# Autodesk Inventor assembly: supportForWinch
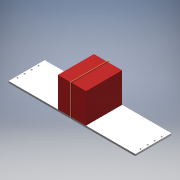
[picture p0: Inventor's stored thumbnail of the model, 180x180]
Saved by Autodesk Inventor 2018.2 (Build 222227000, 227)
## iProperties
Created: 2018-01-10
Part Number: supportForWinch
Document SubType Name: Assembly
Designer: steele
Author: steele
## Documents named in this file (3)
- D:\snobotics\CAD-Development\robSteele\2018-FRC\supportForWinch.iam
- D:\snobotics\CAD-Development\robSteele\2018-FRC\AluminumPlateForWinch.ipt
- D:\snobotics\CAD-Development\robSteele\2018-FRC\WinchVolume.ipt
## Components (2 placed, 2 different names)
1. AluminumPlateForWinch:1 — Mate:6, Flush:3
2. WinchVolume:1 — Mate:6, Flush:3
## Relationships (2: Mate 1, Flush 1)
- Mate:6: AluminumPlateForWinch:1 ↔ WinchVolume:1
- Flush:3: AluminumPlateForWinch:1 ↔ WinchVolume:1
